# Autodesk Inventor assembly: MotorBlockModelisme
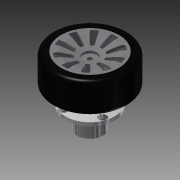
[picture p0: Inventor's stored thumbnail of the model, 180x180]
Saved by Autodesk Inventor 2014 SP1 (Build 180222100, 222)
## iProperties
Created: 2015-04-18
Part Number: MotorBlockModelisme
Document SubType Name: Assembly
Designer: david
Author: david
## Documents named in this file (4)
- C:\Users\asus\Documents\Autodesk\Projects\AUSBEEDone\Components\Motors\MotorBlockModelling.iam
- C:\Users\asus\Documents\Autodesk\Projects\AUSBEEDone\Components\Motors\Motor.iam
- C:\Users\asus\Documents\Autodesk\Projects\AUSBEEDone\Components\Modelling\Hub_Hex_12mm.ipt
- C:\Users\asus\Documents\Autodesk\Projects\AUSBEEDone\Components\Modelling\ModellingWheel_65mm.ipt
## Components (3 placed, 3 different names)
1. Motor:1 [sub-assembly] — Mate:1, Mate:2
2. ModellingWheel_65mm:1 — Angle:1, Mate:8, Mate:9
3. Hub_Hex_12mm:1 — Mate:1, Mate:2, Angle:1, Mate:8, Mate:9
## Relationships (5: Mate 4, Angle 1)
- Mate:1: Motor:1 ↔ Hub_Hex_12mm:1
- Mate:2: Motor:1 ↔ Hub_Hex_12mm:1
- Angle:1 (180 deg): ModellingWheel_65mm:1 ↔ Hub_Hex_12mm:1
- Mate:8: ModellingWheel_65mm:1 ↔ Hub_Hex_12mm:1
- Mate:9: ModellingWheel_65mm:1 ↔ Hub_Hex_12mm:1
